# Autodesk Inventor assembly: nc_nhk10
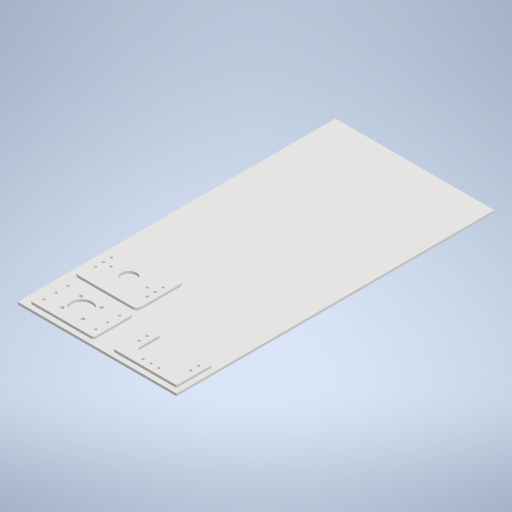
[picture p0: Inventor's stored thumbnail of the model, 512x512]
Saved by Autodesk Inventor 2023 (Build 270158000, 158)
## iProperties
Created: 2022-04-22
Part Number: nc_nhk10
Document SubType Name: Assembly
Designer: yuta
Author: yuta
## Documents named in this file (6)
- C:\Users\yuta\Documents\NHK\nc_nhk10.iam
- C:\Users\yuta\Documents\NHK\NC.port.ipt
- C:\Users\yuta\Documents\NHK\射出_固定1.ipt
- C:\Users\yuta\Documents\NHK\射出_モーター固定1.ipt
- E:\Part1.ipt
- C:\Users\yuta\Documents\NHK\射出_エンコーダー固定2.ipt
## Components (5 placed, 5 different names)
1. NC.port:1 — メイト:1, フラッシュ:1, メイト:2, フラッシュ:2, フラッシュ:3, メイト:3, フラッシュ:4, メイト:5, フラッシュ:5
2. 射出_固定1:2 — メイト:2, フラッシュ:2, フラッシュ:3
3. 射出_モーター固定1:1 — メイト:1, フラッシュ:1, メイト:4, メイト:6
4. Part1:1 — メイト:3, メイト:4, フラッシュ:4
5. 射出_エンコーダー固定2:1 — メイト:5, フラッシュ:5, メイト:6
## Relationships (11: Mate 6, Flush 5)
- メイト:1 [Mate]: NC.port:1 ↔ 射出_モーター固定1:1
- フラッシュ:1 [Flush] (6 mm): NC.port:1 ↔ 射出_モーター固定1:1
- メイト:2 [Mate]: NC.port:1 ↔ 射出_固定1:2
- フラッシュ:2 [Flush] (6 mm): NC.port:1 ↔ 射出_固定1:2
- フラッシュ:3 [Flush] (6 mm): NC.port:1 ↔ 射出_固定1:2
- メイト:3 [Mate]: NC.port:1 ↔ Part1:1
- メイト:4 [Mate] (8 mm): 射出_モーター固定1:1 ↔ Part1:1
- フラッシュ:4 [Flush] (6 mm): NC.port:1 ↔ Part1:1
- メイト:5 [Mate]: NC.port:1 ↔ 射出_エンコーダー固定2:1
- フラッシュ:5 [Flush] (6 mm): NC.port:1 ↔ 射出_エンコーダー固定2:1
- メイト:6 [Mate] (8 mm): 射出_モーター固定1:1 ↔ 射出_エンコーダー固定2:1
